# Autodesk Inventor assembly: HipRight
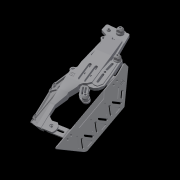
[picture p0: Inventor's stored thumbnail of the model, 180x180]
Saved by Autodesk Inventor 2015 (Build 190159000, 159)
## iProperties
Created: 2014-09-01
Part Number: HipRight
Document SubType Name: Assembly
Designer: Inventor
Mass: 809.946 g
Surface Area: 1272.46 cm^2
Volume: 359.464 cm^3
Density: 2.2532 g/cm^3
Author: Inventor
## Documents named in this file (7)
- D:\Desktop\elysium-max-exoskeleton\src\Assemblies\HipRight.iam
- D:\Desktop\elysium-max-exoskeleton\src\SpacerShort.ipt
- D:\Desktop\elysium-max-exoskeleton\src\HipRight.ipt
- D:\Desktop\elysium-max-exoskeleton\src\HipTopConnectorRight.ipt
- D:\Desktop\elysium-max-exoskeleton\src\HipBottomConnectorRight.ipt
- D:\Desktop\elysium-max-exoskeleton\src\HipShockPlateRight.ipt
- D:\Desktop\elysium-max-exoskeleton\src\HipPistonConnectorRight.ipt
## Components (8 placed, 6 different names)
1. HipRight:1 — Mate:27, Mate:39, Mate:40, Mate:48, Mate:49, Mate:50, Mate:51, Mate:54, Mate:56
2. HipTopConnectorRight:1 — Mate:46, Mate:47, Angle:1, Mate:48
3. HipBottomConnectorRight:1 — Mate:27, Mate:39, Mate:40, Mate:42
4. HipShockPlateRight:1 — Mate:42, Mate:46, Mate:47, Angle:1
5. HipPistonConnectorRight:1 — Mate:55, Mate:56
6. SpacerShort:4 — Mate:51, Mate:54
7. SpacerShort:5 — Mate:49, Mate:50
8. SpacerShort:6 — Mate:55
## Relationships (14: Mate 13, Angle 1)
- Mate:27: HipRight:1 ↔ HipBottomConnectorRight:1
- Mate:39: HipRight:1 ↔ HipBottomConnectorRight:1
- Mate:40: HipRight:1 ↔ HipBottomConnectorRight:1
- Mate:42: HipBottomConnectorRight:1 ↔ HipShockPlateRight:1
- Mate:46: HipTopConnectorRight:1 ↔ HipShockPlateRight:1
- Mate:47: HipTopConnectorRight:1 ↔ HipShockPlateRight:1
- Angle:1 (90 deg): HipTopConnectorRight:1 ↔ HipShockPlateRight:1
- Mate:48: HipRight:1 ↔ HipTopConnectorRight:1
- Mate:49: HipRight:1 ↔ SpacerShort:5
- Mate:50: HipRight:1 ↔ SpacerShort:5
- Mate:51: HipRight:1 ↔ SpacerShort:4
- Mate:54: HipRight:1 ↔ SpacerShort:4
- Mate:55: HipPistonConnectorRight:1 ↔ SpacerShort:6
- Mate:56: HipRight:1 ↔ HipPistonConnectorRight:1
